# Autodesk Inventor assembly: Mecanum_Assembly
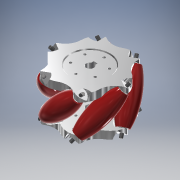
[picture p0: Inventor's stored thumbnail of the model, 180x180]
Saved by Autodesk Inventor 2018 (Build 220112000, 112)
## iProperties
Created: 2017-09-05
Part Number: Mecanum_Assembly
Document SubType Name: Assembly
Designer: P136265
Author: P136265
## Documents named in this file (6)
- C:\Users\P136265\Documents\mecanum-cad\Mecanum_Assembly.iam
- C:\Users\P136265\Documents\mecanum-cad\roller 8-19-6 bearing.ipt
- C:\Users\P136265\Documents\Inventor\Content Center Files\R2018\en-US\DIN 625 SKF(4)\DIN 625 SKF - SKF 619_8-2Z.ipt
- C:\Users\P136265\Documents\mecanum-cad\MecanumShaft.ipt
- C:\Users\P136265\Documents\mecanum-cad\PE_Sleeve.ipt
- C:\Users\P136265\Documents\mecanum-cad\CheekPlate.ipt
## Components (32 placed, 5 different names)
1. CheekPlate:1 — Angle:4, Mate:5, Mate:6, Angle:5
2. CheekPlate:2 — Angle:5, Angle:6, Mate:7, Mate:8
3. roller 8-19-6 bearing:1 — Mate:1, Angle:1, Mate:2
4. roller 8-19-6 bearing:2 — Angle:4, Mate:5
5. roller 8-19-6 bearing:3 — Insert:1, Insert:2
6. roller 8-19-6 bearing:4 — Angle:2, Mate:3, Mate:4, Angle:6, Mate:7, Mate:8
7. roller 8-19-6 bearing:5
8. roller 8-19-6 bearing:6
9. DIN 625 SKF- with two Z shields SKF 619/8-2Z:1 — Insert:1
10. DIN 625 SKF- with two Z shields SKF 619/8-2Z:3
11. DIN 625 SKF- with two Z shields SKF 619/8-2Z:4
12. DIN 625 SKF- with two Z shields SKF 619/8-2Z:5
13. DIN 625 SKF- with two Z shields SKF 619/8-2Z:6
14. DIN 625 SKF- with two Z shields SKF 619/8-2Z:7
15. DIN 625 SKF- with two Z shields SKF 619/8-2Z:2 — Insert:2
16. DIN 625 SKF- with two Z shields SKF 619/8-2Z:8 — Flush:1
17. DIN 625 SKF- with two Z shields SKF 619/8-2Z:9
18. DIN 625 SKF- with two Z shields SKF 619/8-2Z:10
19. DIN 625 SKF- with two Z shields SKF 619/8-2Z:11
20. DIN 625 SKF- with two Z shields SKF 619/8-2Z:12
21. MecanumShaft:1 — Angle:2, Mate:3, Flush:1, Angle:3
22. MecanumShaft:2
23. MecanumShaft:3
24. MecanumShaft:4
25. MecanumShaft:5
26. MecanumShaft:6 — Mate:6
27. PE_Sleeve:1 — Angle:3, Mate:4
28. PE_Sleeve:2
29. PE_Sleeve:3
30. PE_Sleeve:4
31. PE_Sleeve:5
32. PE_Sleeve:6
## Component patterns: (6 elements, first: roller 8-19-6 bearing:1), (6 elements, first: DIN 625 SKF- with two Z shields SKF 619/8-2Z:1), (6 elements, first: DIN 625 SKF- with two Z shields SKF 619/8-2Z:2), (6 elements, first: MecanumShaft:1), (6 elements, first: PE_Sleeve:1)
## Relationships (17: Mate 8, Angle 6, Insert 2, Flush 1)
- Mate:1 (75 mm): roller 8-19-6 bearing:1
- Angle:1 (45 deg): roller 8-19-6 bearing:1
- Mate:2: roller 8-19-6 bearing:1
- Insert:1: roller 8-19-6 bearing:3 ↔ DIN 625 SKF- with two Z shields SKF 619/8-2Z:1
- Insert:2: roller 8-19-6 bearing:3 ↔ DIN 625 SKF- with two Z shields SKF 619/8-2Z:2
- Angle:2 (0 deg): roller 8-19-6 bearing:4 ↔ MecanumShaft:1
- Mate:3: roller 8-19-6 bearing:4 ↔ MecanumShaft:1
- Flush:1 (-20 mm): DIN 625 SKF- with two Z shields SKF 619/8-2Z:8 ↔ MecanumShaft:1
- Angle:3 (0 deg): MecanumShaft:1 ↔ PE_Sleeve:1
- Mate:4: roller 8-19-6 bearing:4 ↔ PE_Sleeve:1
- Angle:4 (0 deg): CheekPlate:1 ↔ roller 8-19-6 bearing:2
- Mate:5 (1 mm): CheekPlate:1 ↔ roller 8-19-6 bearing:2
- Mate:6: CheekPlate:1 ↔ MecanumShaft:6
- Angle:5 (0 deg): CheekPlate:1 ↔ CheekPlate:2
- Angle:6 (0 deg): CheekPlate:2 ↔ roller 8-19-6 bearing:4
- Mate:7 (1 mm): CheekPlate:2 ↔ roller 8-19-6 bearing:4
- Mate:8: CheekPlate:2 ↔ roller 8-19-6 bearing:4
